# Autodesk Inventor assembly: smartPowerStrip
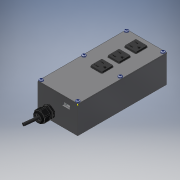
[picture p0: Inventor's stored thumbnail of the model, 180x180]
Saved by Autodesk Inventor 2018 (Build 220112000, 112)
## iProperties
Created: 2018-02-08
Part Number: smartPowerStrip
Document SubType Name: Assembly
Designer: artur
Author: artur
## Documents named in this file (10)
- C:\Users\artur\Documents\projects\smartPowerStrip\CAD\Mechanical\smartPowerStrip.iam
- C:\Users\artur\Documents\projects\smartPowerStrip\CAD\Mechanical\Housing Rev 3.ipt
- C:\Users\artur\Documents\projects\smartPowerStrip\CAD\Mechanical\Cover Rev 4.ipt
- C:\Users\artur\Documents\projects\smartPowerStrip\CAD\Mechanical\ESP8266_ThingDevBoard.ipt
- C:\Users\artur\Documents\projects\smartPowerStrip\CAD\Mechanical\dimmerModule.ipt
- C:\Users\artur\Documents\projects\smartPowerStrip\CAD\Mechanical\QUALTEK 738W-X201.ipt
- C:\Users\artur\Documents\projects\smartPowerStrip\CAD\Mechanical\AC2DC_real.iam
- C:\Users\artur\Documents\projects\smartPowerStrip\CAD\Mechanical\wire.ipt
- C:\Users\artur\Documents\projects\smartPowerStrip\CAD\Mechanical\AIS2018\CD13NA-BK.iam
- C:\Users\artur\Documents\projects\smartPowerStrip\CAD\Mechanical\PanHeadCrossRecessedScrew_M4x10.ipt
## Components (16 placed, 9 different names)
1. Housing Rev 3:1 — Mate:1, Mate:2, Mate:3, Mate:13, Mate:14, Mate:15, Mate:16, Mate:17, Mate:18, Mate:19, Mate:21, Mate:22, Mate:23, Mate:24, Mate:25, Mate:26, Mate:27, Mate:28, Mate:29
2. Cover Rev 4:1 — Mate:1, Mate:4, Mate:5, Mate:6, Mate:7, Mate:8, Mate:9, Mate:10, Mate:11, Mate:12, Mate:13, Mate:30, Mate:31, Mate:32, Mate:33, Mate:34, Mate:35
3. ESP8266_ThingDevBoard:1 — Mate:2, Mate:14, Mate:15
4. dimmerModule:1 — Mate:3, Mate:16
5. QUALTEK 738W-X201:1 — Mate:4, Mate:11, Mate:12
6. QUALTEK 738W-X201:2 — Mate:5, Mate:9, Mate:10
7. QUALTEK 738W-X201:3 — Mate:6, Mate:7, Mate:8
8. AC2DC_real:1 [sub-assembly] — Mate:17, Mate:18
9. wire:1 — Mate:19, Mate:23
10. CD13NA-BK:1 [sub-assembly] — Mate:21, Mate:22
11. PanHeadCrossRecessedScrew_M4x10:1 — Mate:29, Mate:30
12. PanHeadCrossRecessedScrew_M4x10:2 — Mate:28, Mate:32
13. PanHeadCrossRecessedScrew_M4x10:3 — Mate:27, Mate:35
14. PanHeadCrossRecessedScrew_M4x10:4 — Mate:26, Mate:34
15. PanHeadCrossRecessedScrew_M4x10:5 — Mate:25, Mate:33
16. PanHeadCrossRecessedScrew_M4x10:7 — Mate:24, Mate:31
## Relationships (34: Mate 34)
- Mate:1: Housing Rev 3:1 ↔ Cover Rev 4:1
- Mate:2 (40.64 mm): Housing Rev 3:1 ↔ ESP8266_ThingDevBoard:1
- Mate:3 (0.635 mm): Housing Rev 3:1 ↔ dimmerModule:1
- Mate:4: Cover Rev 4:1 ↔ QUALTEK 738W-X201:1
- Mate:5: Cover Rev 4:1 ↔ QUALTEK 738W-X201:2
- Mate:6: Cover Rev 4:1 ↔ QUALTEK 738W-X201:3
- Mate:7 (0.127 mm): Cover Rev 4:1 ↔ QUALTEK 738W-X201:3
- Mate:8 (3.81 mm): Cover Rev 4:1 ↔ QUALTEK 738W-X201:3
- Mate:9: Cover Rev 4:1 ↔ QUALTEK 738W-X201:2
- Mate:10 (3.81 mm): Cover Rev 4:1 ↔ QUALTEK 738W-X201:2
- Mate:11: Cover Rev 4:1 ↔ QUALTEK 738W-X201:1
- Mate:12 (3.81 mm): Cover Rev 4:1 ↔ QUALTEK 738W-X201:1
- Mate:13: Housing Rev 3:1 ↔ Cover Rev 4:1
- Mate:14 (6.35 mm): Housing Rev 3:1 ↔ ESP8266_ThingDevBoard:1
- Mate:15 (-6.35 mm): Housing Rev 3:1 ↔ ESP8266_ThingDevBoard:1
- Mate:16 (6.35 mm): Housing Rev 3:1 ↔ dimmerModule:1
- Mate:17 (12.7 mm): Housing Rev 3:1 ↔ AC2DC_real:1
- Mate:18 (12.7 mm): Housing Rev 3:1 ↔ AC2DC_real:1
- Mate:19 (12.7 mm): Housing Rev 3:1 ↔ wire:1
- Mate:21: Housing Rev 3:1 ↔ CD13NA-BK:1
- Mate:22: Housing Rev 3:1 ↔ CD13NA-BK:1
- Mate:23: Housing Rev 3:1 ↔ wire:1
- Mate:24: Housing Rev 3:1 ↔ PanHeadCrossRecessedScrew_M4x10:7
- Mate:25: Housing Rev 3:1 ↔ PanHeadCrossRecessedScrew_M4x10:5
- Mate:26: Housing Rev 3:1 ↔ PanHeadCrossRecessedScrew_M4x10:4
- Mate:27: Housing Rev 3:1 ↔ PanHeadCrossRecessedScrew_M4x10:3
- Mate:28: Housing Rev 3:1 ↔ PanHeadCrossRecessedScrew_M4x10:2
- Mate:29: Housing Rev 3:1 ↔ PanHeadCrossRecessedScrew_M4x10:1
- Mate:30: Cover Rev 4:1 ↔ PanHeadCrossRecessedScrew_M4x10:1
- Mate:31: Cover Rev 4:1 ↔ PanHeadCrossRecessedScrew_M4x10:7
- Mate:32: Cover Rev 4:1 ↔ PanHeadCrossRecessedScrew_M4x10:2
- Mate:33: Cover Rev 4:1 ↔ PanHeadCrossRecessedScrew_M4x10:5
- Mate:34: Cover Rev 4:1 ↔ PanHeadCrossRecessedScrew_M4x10:4
- Mate:35: Cover Rev 4:1 ↔ PanHeadCrossRecessedScrew_M4x10:3
